# Autodesk Inventor assembly: DC_convertor
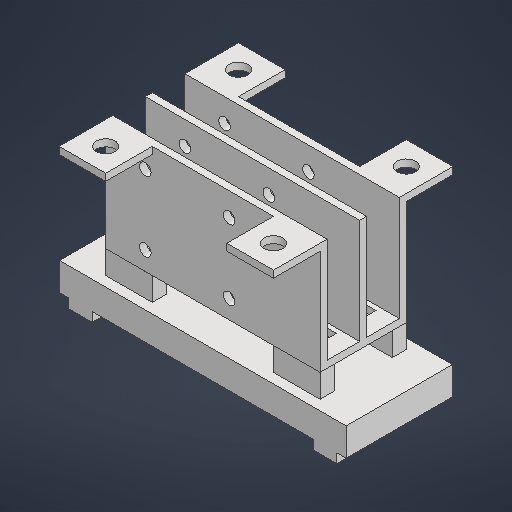
[picture p0: Inventor's stored thumbnail of the model, 512x512]
Saved by Autodesk Inventor 2026.1 (Build 301233020, 233B)
## iProperties
Created: 2025-11-26
Part Number: DC_convertor
Document SubType Name: Assembly
Designer: jaewook
Author: jaewook
## Documents named in this file (4)
- C:\Users\kjh19\Documents\Inventor\project\turrte_projict_v2\DC_convertor.iam
- C:\Users\kjh19\Documents\Inventor\project\turrte_projict_v2\dc_convertor.ipt
- C:\Users\kjh19\Documents\Inventor\project\turrte_projict_v2\convertor_base.ipt
- C:\Users\kjh19\Documents\Inventor\project\turrte_projict_v2\converter2.ipt
## Components (3 placed, 3 different names)
1. dc_convertor:1
2. convertor_base:1 — 메이트:1, 메이트:2
3. converter2:1 — 메이트:1, 메이트:2
## Relationships (2: Mate 2)
- 메이트:1 [Mate]: convertor_base:1 ↔ converter2:1
- 메이트:2 [Mate]: convertor_base:1 ↔ converter2:1
